# Autodesk Inventor assembly: Assembly1
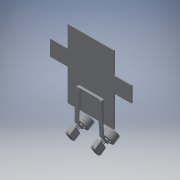
[picture p0: Inventor's stored thumbnail of the model, 180x180]
Saved by Autodesk Inventor 2019 (Build 230136000, 136)
## iProperties
Created: 2019-10-15
Part Number: Assembly1
Document SubType Name: Assembly
Designer: User
Author: User
## Documents named in this file (3)
- C:\Robotics\CAD\2019-20_CAD\Collection\Assembly1.iam
- C:\Robotics\CAD\2019-20_CAD\Collection\20Gen2PlatePart .ipt
- C:\Robotics\CAD\2019-20_CAD\Collection\U assembly.iam
## Components (2 placed, 2 different names)
1. 20Gen2PlatePart :1 — Mate:1, Flush:1, Flush:2
2. U assembly:1 [sub-assembly] — Mate:1, Flush:1, Flush:2
## Relationships (3: Flush 2, Mate 1)
- Mate:1: 20Gen2PlatePart :1 ↔ U assembly:1
- Flush:1 (12.7 mm): 20Gen2PlatePart :1 ↔ U assembly:1
- Flush:2 (50.8 mm): 20Gen2PlatePart :1 ↔ U assembly:1
